# Autodesk Inventor assembly: Panel asm
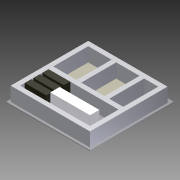
[picture p0: Inventor's stored thumbnail of the model, 180x180]
Saved by Autodesk Inventor 2011 (Build 150239000, 239)
## iProperties
Created: 2013-11-27
Part Number: Panel asm
Document SubType Name: Assembly
Designer: Devon
Author: Devon
## Documents named in this file (9)
- C:\Users\Devon\Dropbox\ELEC 4497 - Senior Design\Design\Electrical\Panel asm.iam
- C:\Users\Devon\Dropbox\ELEC 4497 - Senior Design\Design\Electrical\panel.ipt
- C:\Users\Devon\Dropbox\ELEC 4497 - Senior Design\Design\Electrical\17in wire duct.ipt
- C:\Users\Devon\Dropbox\ELEC 4497 - Senior Design\Design\Electrical\15in wire duct.ipt
- C:\Users\Devon\Dropbox\ELEC 4497 - Senior Design\Design\Electrical\4x6.5 PCB.ipt
- C:\Users\Devon\Dropbox\ELEC 4497 - Senior Design\Design\Electrical\7.5in wire duct.ipt
- C:\Users\Devon\Dropbox\ELEC 4497 - Senior Design\Design\Electrical\2x6.5 PCB.ipt
- C:\Users\Devon\Dropbox\ELEC 4497 - Senior Design\Design\Electrical\Stepper Drive.ipt
- C:\Users\Devon\Dropbox\ELEC 4497 - Senior Design\Design\Electrical\Power Suplply.ipt
## Components (15 placed, 8 different names)
1. panel:1 — Mate:1, Mate:2, Flush:1, Flush:2, Flush:3, Flush:4, Mate:3, Mate:4, Mate:5, Mate:9, Mate:10, Mate:15, Mate:19, Mate:22, Mate:25, Mate:26, Mate:27, Mate:28
2. 17in wire duct:1 — Mate:1, Flush:3, Flush:4, Mate:6, Flush:5, Mate:7, Flush:6, Mate:8, Mate:13, Mate:29, Mate:31, Mate:33
3. 17in wire duct:3 — Mate:2, Flush:1, Flush:2, Mate:24, Mate:36
4. 15in wire duct:1 — Mate:5, Mate:6, Flush:5, Mate:35
5. 15in wire duct:2 — Mate:4, Mate:8, Mate:14, Mate:30
6. 15in wire duct:3 — Mate:3, Mate:7, Flush:6, Mate:11, Mate:12, Mate:16, Mate:20, Mate:23
7. 4x6.5 PCB:1 — Mate:9, Mate:12, Mate:13, Mate:17
8. 4x6.5 PCB:2 — Mate:10, Mate:11, Mate:14, Mate:18, Mate:21
9. 7.5in wire duct:1 — Mate:15, Mate:16, Mate:17, Mate:18
10. 7.5in wire duct:2 — Mate:19, Mate:20, Mate:21
11. 2x6.5 PCB:1 — Mate:22, Mate:23, Mate:24
12. Stepper Drive:1 — Mate:26, Mate:31, Mate:32, Mate:34
13. Stepper Drive:2 — Mate:27, Mate:33, Mate:34
14. Stepper Drive:3 — Mate:28, Mate:29, Mate:30, Mate:32
15. Power Suplply:1 — Mate:25, Mate:35, Mate:36
## Relationships (42: Mate 36, Flush 6)
- Mate:1: panel:1 ↔ 17in wire duct:1
- Mate:2: panel:1 ↔ 17in wire duct:3
- Flush:1 (12.7 mm): panel:1 ↔ 17in wire duct:3
- Flush:2 (12.7 mm): panel:1 ↔ 17in wire duct:3
- Flush:3 (12.7 mm): panel:1 ↔ 17in wire duct:1
- Flush:4 (12.7 mm): panel:1 ↔ 17in wire duct:1
- Mate:3: panel:1 ↔ 15in wire duct:3
- Mate:4: panel:1 ↔ 15in wire duct:2
- Mate:5: panel:1 ↔ 15in wire duct:1
- Mate:6: 17in wire duct:1 ↔ 15in wire duct:1
- Flush:5: 17in wire duct:1 ↔ 15in wire duct:1
- Mate:7: 17in wire duct:1 ↔ 15in wire duct:3
- Flush:6: 17in wire duct:1 ↔ 15in wire duct:3
- Mate:8: 17in wire duct:1 ↔ 15in wire duct:2
- Mate:9: panel:1 ↔ 4x6.5 PCB:1
- Mate:10: panel:1 ↔ 4x6.5 PCB:2
- Mate:11 (12.7 mm): 15in wire duct:3 ↔ 4x6.5 PCB:2
- Mate:12 (12.7 mm): 15in wire duct:3 ↔ 4x6.5 PCB:1
- Mate:13 (12.7 mm): 17in wire duct:1 ↔ 4x6.5 PCB:1
- Mate:14 (12.7 mm): 15in wire duct:2 ↔ 4x6.5 PCB:2
- Mate:15: panel:1 ↔ 7.5in wire duct:1
- Mate:16: 15in wire duct:3 ↔ 7.5in wire duct:1
- Mate:17 (12.7 mm): 4x6.5 PCB:1 ↔ 7.5in wire duct:1
- Mate:18 (12.7 mm): 4x6.5 PCB:2 ↔ 7.5in wire duct:1
- Mate:19: panel:1 ↔ 7.5in wire duct:2
- Mate:20: 15in wire duct:3 ↔ 7.5in wire duct:2
- Mate:21 (12.7 mm): 4x6.5 PCB:2 ↔ 7.5in wire duct:2
- Mate:22: panel:1 ↔ 2x6.5 PCB:1
- Mate:23 (12.7 mm): 15in wire duct:3 ↔ 2x6.5 PCB:1
- Mate:24 (12.7 mm): 17in wire duct:3 ↔ 2x6.5 PCB:1
- Mate:25: panel:1 ↔ Power Suplply:1
- Mate:26: panel:1 ↔ Stepper Drive:1
- Mate:27: panel:1 ↔ Stepper Drive:2
- Mate:28: panel:1 ↔ Stepper Drive:3
- Mate:29 (12.7 mm): 17in wire duct:1 ↔ Stepper Drive:3
- Mate:30 (12.7 mm): 15in wire duct:2 ↔ Stepper Drive:3
- Mate:31 (12.7 mm): 17in wire duct:1 ↔ Stepper Drive:1
- Mate:32 (12.7 mm): Stepper Drive:1 ↔ Stepper Drive:3
- Mate:33 (12.7 mm): 17in wire duct:1 ↔ Stepper Drive:2
- Mate:34 (12.7 mm): Stepper Drive:1 ↔ Stepper Drive:2
- Mate:35 (12.7 mm): 15in wire duct:1 ↔ Power Suplply:1
- Mate:36 (12.7 mm): 17in wire duct:3 ↔ Power Suplply:1
